# Autodesk Inventor assembly: BaseAssembly
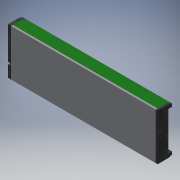
[picture p0: Inventor's stored thumbnail of the model, 180x180]
Saved by Autodesk Inventor 2016 (Build 200138000, 138)
## iProperties
Created: 2015-05-19
Part Number: BaseAssembly
Document SubType Name: Assembly
Designer: Andy
Mass: 20870 g
Surface Area: 13183.8 cm^2
Volume: 4333.01 cm^3
Author: Andy
## Documents named in this file (8)
- C:\Users\jonathan\Desktop\Inverted Pendulum CAD\Base Assembly.iam
- C:\Users\jonathan\Desktop\Inverted Pendulum CAD\Base Front Back Side.ipt
- C:\Users\jonathan\Desktop\Inverted Pendulum CAD\Base Bottom.ipt
- C:\Users\jonathan\Desktop\Inverted Pendulum CAD\Base Left Side.ipt
- C:\Users\jonathan\Desktop\Inverted Pendulum CAD\Base Right Side.ipt
- C:\Users\jonathan\Desktop\Inverted Pendulum CAD\Track.ipt
- C:\Users\jonathan\Desktop\Inverted Pendulum CAD\Base Wire Holder.ipt
- C:\Users\jonathan\Desktop\Inverted Pendulum CAD\Base Magnetic Strip.ipt
## Components (9 placed, 7 different names)
1. Base Bottom:1 — Mate:2, Flush:3, Flush:4, Mate:4, Flush:5, Flush:6, Mate:6, Mate:12, Mate:16, Flush:11, Flush:12, Mate:17, Mate:24
2. Base Right Side:1 — Mate:2, Flush:3, Flush:4, Mate:14, Mate:15, Mate:18
3. Track:1 — Mate:26
4. Base Front Back Side:1 — Flush:6, Mate:6, Mate:13, Mate:15
5. Base Front Back Side:2 — Mate:4, Flush:5, Mate:27
6. Track:2 — Mate:24, Mate:25
7. Base Wire Holder:1 — Mate:12, Mate:13, Mate:14, Mate:19
8. Base Left Side:1 — Mate:16, Flush:11, Flush:12, Mate:25, Mate:26, Mate:27
9. Base Magnetic Strip:1 — Mate:17, Mate:18, Mate:19
## Relationships (21: Mate 15, Flush 6)
- Mate:2: Base Bottom:1 ↔ Base Right Side:1
- Flush:3: Base Bottom:1 ↔ Base Right Side:1
- Flush:4: Base Bottom:1 ↔ Base Right Side:1
- Mate:4: Base Bottom:1 ↔ Base Front Back Side:2
- Flush:5: Base Bottom:1 ↔ Base Front Back Side:2
- Flush:6: Base Bottom:1 ↔ Base Front Back Side:1
- Mate:6: Base Bottom:1 ↔ Base Front Back Side:1
- Mate:12: Base Bottom:1 ↔ Base Wire Holder:1
- Mate:13 (55 mm): Base Front Back Side:1 ↔ Base Wire Holder:1
- Mate:14 (33 mm): Base Right Side:1 ↔ Base Wire Holder:1
- Mate:15: Base Right Side:1 ↔ Base Front Back Side:1
- Mate:16: Base Bottom:1 ↔ Base Left Side:1
- Flush:11: Base Bottom:1 ↔ Base Left Side:1
- Flush:12: Base Bottom:1 ↔ Base Left Side:1
- Mate:17: Base Bottom:1 ↔ Base Magnetic Strip:1
- Mate:18: Base Right Side:1 ↔ Base Magnetic Strip:1
- Mate:19 (31.5 mm): Base Wire Holder:1 ↔ Base Magnetic Strip:1
- Mate:24: Base Bottom:1 ↔ Track:2
- Mate:25 (10 mm): Track:2 ↔ Base Left Side:1
- Mate:26 (10 mm): Track:1 ↔ Base Left Side:1
- Mate:27: Base Front Back Side:2 ↔ Base Left Side:1
